# Autodesk Inventor assembly: P32-5M-15AL
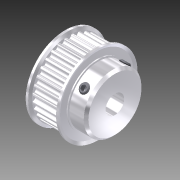
[picture p0: Inventor's stored thumbnail of the model, 180x180]
Saved by Autodesk Inventor 2011 (Build 150239000, 239)
## iProperties
Category: Miscellaneous
Company: Autodesk Inc.
Created: 2008-11-19
Part Number: P32-5M-15AL
Document SubType Name: Assembly
Designer: Autodesk Inc.
Catalog Web Link: http://www.gates.com/catalogs/file_display.cfm?file=SynchronousMetal.pdf&thisPath=gates\catalogs
Description: Sprocket 32 teeth
Vendor: Gates
Mass: 250 g
Surface Area: 140.045 cm^2
Volume: 50.7564 cm^3
Author: Autodesk Inc.
## Documents named in this file (3)
- R:\2012\Inventor\vkop\All_Miscellaneous\SupportingSprocket_Gates_P32-5M-15AL.iam
- R:\2012\Inventor\vkop\All_Miscellaneous\SupportingSprocket_Gates_P32-5M-15AL.ipt
- R:\2012\Inventor\vkop\All_Miscellaneous\ANSI B18.3 - 1_4-20 UNC - 0.625(24).ipt
## Components (3 placed, 2 different names)
1. SupportingSprocket_Gates_P32-5M-15AL:1 — Mate:1, Mate:2
2. Hexagon Socket Set Screw - Flat Point - Inch 1/4-20 UNC x 0.625:1 — Mate:1
3. Hexagon Socket Set Screw - Flat Point - Inch 1/4-20 UNC x 0.625:2 — Mate:2
## Relationships (2: Mate 2)
- Mate:1: SupportingSprocket_Gates_P32-5M-15AL:1 ↔ Hexagon Socket Set Screw - Flat Point - Inch 1/4-20 UNC x 0.625:1
- Mate:2: SupportingSprocket_Gates_P32-5M-15AL:1 ↔ Hexagon Socket Set Screw - Flat Point - Inch 1/4-20 UNC x 0.625:2
